# Autodesk Inventor assembly: Ensamble NotAFarmBot2
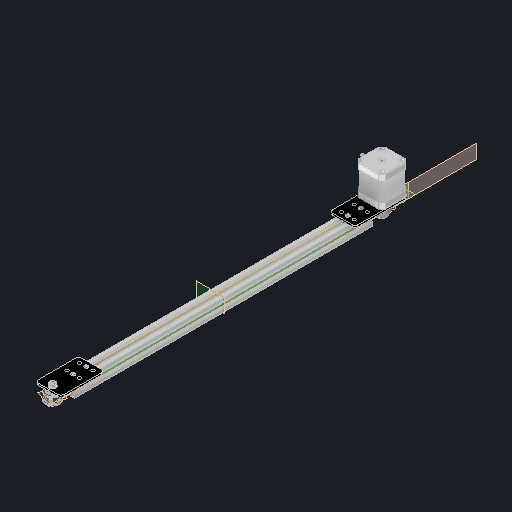
[picture p0: Inventor's stored thumbnail of the model, 512x512]
Saved by Autodesk Inventor 2024 (Build 280153000, 153)
## iProperties
Created: 2020-07-22
Part Number: Ensamble NotAFarmBot2
Document SubType Name: Assembly
Designer: juanp
Mass: 1932.13 g
Surface Area: 7509.2 cm^2
Volume: 1044.57 cm^3
Density: 1.84968 g/cm^3
Author: juanp
## Documents named in this file (17)
- C:\Users\juanp\OneDrive - Universidad de los andes\Uniandes\Robocol\SyE - EVA + RAMSES\EVA\Recursos\Actuador Lineal\Actuador Lineal (sin carro).iam
- C:\Users\juanp\OneDrive - Universidad de los andes\Uniandes\Robocol\SyE - EVA + RAMSES\EVA\Recursos\Actuador Lineal\Partes\VSLOT 2020 Extrusion.ipt
- C:\Users\juanp\OneDrive - Universidad de los andes\Uniandes\Robocol\SyE - EVA + RAMSES\EVA\Recursos\Actuador Lineal\Tornillos-Arandelas-Tuercas-Espaciadores\Double Tee Nut.ipt
- C:\Users\juanp\OneDrive - Universidad de los andes\Uniandes\Robocol\SyE - EVA + RAMSES\EVA\Recursos\Actuador Lineal\Partes\GT2_30T_5_6.ipt
- C:\Users\juanp\OneDrive - Universidad de los andes\Uniandes\Robocol\SyE - EVA + RAMSES\EVA\Recursos\Actuador Lineal\Partes\Idler Pulley Plate.ipt
- C:\Users\juanp\OneDrive - Universidad de los andes\Uniandes\Robocol\SyE - EVA + RAMSES\EVA\Recursos\Actuador Lineal\Partes\Motor Mount Plate Nema 17.ipt
- C:\Users\juanp\OneDrive - Universidad de los andes\Uniandes\Robocol\SyE - EVA + RAMSES\EVA\Recursos\Actuador Lineal\Partes\M1173041- NEMA 17.ipt
- C:\Users\juanp\OneDrive - Universidad de los andes\Uniandes\Robocol\SyE - EVA + RAMSES\EVA\Recursos\Actuador Lineal\Tornillos-Arandelas-Tuercas-Espaciadores\3mm Spacer.ipt
- C:\Users\juanp\OneDrive - Universidad de los andes\Uniandes\Robocol\SyE - EVA + RAMSES\EVA\Recursos\Actuador Lineal\Partes\Ball Bearing 625 2RS 5x16x5.ipt
- C:\Users\juanp\OneDrive - Universidad de los andes\Uniandes\Robocol\SyE - EVA + RAMSES\EVA\Recursos\Actuador Lineal\Tornillos-Arandelas-Tuercas-Espaciadores\1mm 5mm shim.ipt
- C:\Users\juanp\OneDrive - Universidad de los andes\Uniandes\Robocol\SyE - EVA + RAMSES\EVA\Recursos\Actuador Lineal\Tornillos-Arandelas-Tuercas-Espaciadores\Nylon Spacer 1_8th.ipt
- C:\Users\juanp\OneDrive - Universidad de los andes\Uniandes\Robocol\SyE - EVA + RAMSES\EVA\Recursos\Actuador Lineal\Partes\idler pulley.ipt
- C:\Users\juanp\OneDrive - Universidad de los andes\Uniandes\Robocol\SyE - EVA + RAMSES\EVA\Recursos\Actuador Lineal\Tornillos-Arandelas-Tuercas-Espaciadores\M5 Nylock.ipt
- C:\Users\juanp\OneDrive - Universidad de los andes\Uniandes\Robocol\SyE - EVA + RAMSES\EVA\Recursos\Actuador Lineal\Tornillos-Arandelas-Tuercas-Espaciadores\M5x25 low profile screw.ipt
- C:\Users\juanp\Documents\Inventor\Content Center Files\R2020\en-US\ANSI B18.3.1M(1)\ANSI B18.3.1M - M3x0.5 x 8(2).ipt
- C:\Users\juanp\Documents\Inventor\Content Center Files\R2020\en-US\ANSI B18.22 M\ANSI B18.22M - 3 N.ipt
- C:\Users\juanp\Documents\Inventor\Content Center Files\R2020\en-US\ANSI B18.3.4M(2)\ANSI B18.3.4M - M3 x 0.5 x 8(1).ipt
## Components (27 placed, 16 different names)
1. VSLOT 2020 Extrusion:1 — Mate:85, Mate:87, Mate:88, Angle:16, Mate:98, Mate:99, Angle:18, Mate:101, Mate:185, Angle:24, Flush:3, Mate:196, Mate:197, Flush:4, Flush:5
2. Double Tee Nut:1 — Mate:98, Mate:99, Angle:18, Mate:198, Mate:199, Flush:5
3. Double Tee Nut:2 — Mate:85, Mate:87, Angle:16, Mate:200, Mate:201, Flush:4
4. GT2_30T_5_6:2 — Mate:35, Mate:107
5. Idler Pulley Plate:1 — Mate:88, Mate:95, Mate:97, Angle:17, Mate:200, Mate:201, Mate:206, Mate:221, Mate:222
6. Motor Mount Plate Nema 17:1 — Mate:12, Mate:13, Angle:4, Mate:101, Angle:24, Mate:198, Mate:199, Mate:214, Mate:218, Mate:219, Mate:220
7. M1173041- NEMA 17:1 — Mate:12, Mate:13, Angle:4, Mate:107, Mate:213, Mate:215, Mate:216, Mate:217
8. Ball Bearing 625 2RS 5x16x5:1 — Mate:22, Mate:23, Mate:24, Mate:26, Mate:32, Mate:202
9. Ball Bearing 625 2RS 5x16x5:2 — Mate:21, Mate:25, Mate:207
10. 1mm 5mm shim:1 — Mate:47, Mate:97, Mate:205
11. Nylon Spacer 1_8th:1 — Mate:23, Mate:24, Mate:25
12. idler pulley:1 — Mate:21, Mate:22, Mate:26, Mate:35
13. 3mm Spacer:1 — Mate:32, Mate:95, Mate:203
14. M5 Nylock:1 — Mate:47, Angle:17, Mate:204
15. M5x25 low profile screw:1 — Mate:202, Mate:203, Mate:204, Mate:205, Mate:206, Mate:207
16. Broached Socket Head Cap Screw - Metric M3x0.5 x 8:1 — Mate:211, Flush:7, Flush:8, Mate:217
17. Broached Socket Head Cap Screw - Metric M3x0.5 x 8:2 — Mate:210, Flush:8, Mate:212, Mate:216
18. Broached Socket Head Cap Screw - Metric M3x0.5 x 8:3 — Mate:208, Flush:6, Mate:213
19. Broached Socket Head Cap Screw - Metric M3x0.5 x 8:4 — Mate:209, Flush:6, Flush:7, Mate:215
20. Plain Washer (Metric) 3 N:1 — Mate:209, Flush:10, Flush:11, Mate:212, Mate:214
21. Plain Washer (Metric) 3 N:2 — Mate:210, Flush:9
22. Plain Washer (Metric) 3 N:3 — Mate:208, Flush:11
23. Plain Washer (Metric) 3 N:4 — Mate:211, Flush:9, Flush:10
24. Forged Hexagon Socket Button Head Cap Screw - Metric M3 x 0.5 x 8:1 — Flush:12, Mate:222
25. Forged Hexagon Socket Button Head Cap Screw - Metric M3 x 0.5 x 8:2 — Flush:12, Flush:13, Mate:221
26. Forged Hexagon Socket Button Head Cap Screw - Metric M3 x 0.5 x 8:3 — Flush:13, Flush:14, Mate:220
27. Forged Hexagon Socket Button Head Cap Screw - Metric M3 x 0.5 x 8:4 — Flush:14, Mate:218, Mate:219
## Relationships (65: Mate 48, Flush 12, Angle 5)
- Mate:12: Motor Mount Plate Nema 17:1 ↔ M1173041- NEMA 17:1
- Mate:13: Motor Mount Plate Nema 17:1 ↔ M1173041- NEMA 17:1
- Angle:4 (0 deg): Motor Mount Plate Nema 17:1 ↔ M1173041- NEMA 17:1
- Mate:21: Ball Bearing 625 2RS 5x16x5:2 ↔ idler pulley:1
- Mate:22: Ball Bearing 625 2RS 5x16x5:1 ↔ idler pulley:1
- Mate:23: Ball Bearing 625 2RS 5x16x5:1 ↔ Nylon Spacer 1_8th:1
- Mate:24: Ball Bearing 625 2RS 5x16x5:1 ↔ Nylon Spacer 1_8th:1
- Mate:25: Ball Bearing 625 2RS 5x16x5:2 ↔ Nylon Spacer 1_8th:1
- Mate:26: Ball Bearing 625 2RS 5x16x5:1 ↔ idler pulley:1
- Mate:32: Ball Bearing 625 2RS 5x16x5:1 ↔ 3mm Spacer:1
- Mate:35: GT2_30T_5_6:2 ↔ idler pulley:1
- Mate:47: 1mm 5mm shim:1 ↔ M5 Nylock:1
- Mate:85: VSLOT 2020 Extrusion:1 ↔ Double Tee Nut:2
- Mate:87: VSLOT 2020 Extrusion:1 ↔ Double Tee Nut:2
- Mate:88: VSLOT 2020 Extrusion:1 ↔ Idler Pulley Plate:1
- Angle:16 (180 deg): VSLOT 2020 Extrusion:1 ↔ Double Tee Nut:2
- Mate:95: Idler Pulley Plate:1 ↔ 3mm Spacer:1
- Mate:97: Idler Pulley Plate:1 ↔ 1mm 5mm shim:1
- Angle:17 (0 deg): Idler Pulley Plate:1 ↔ M5 Nylock:1
- Mate:98: VSLOT 2020 Extrusion:1 ↔ Double Tee Nut:1
- Mate:99: VSLOT 2020 Extrusion:1 ↔ Double Tee Nut:1
- Angle:18 (0 deg): VSLOT 2020 Extrusion:1 ↔ Double Tee Nut:1
- Mate:101: VSLOT 2020 Extrusion:1 ↔ Motor Mount Plate Nema 17:1
- Mate:107: GT2_30T_5_6:2 ↔ M1173041- NEMA 17:1
- Mate:185: VSLOT 2020 Extrusion:1
- Angle:24 (0 deg): VSLOT 2020 Extrusion:1 ↔ Motor Mount Plate Nema 17:1
- Flush:3: VSLOT 2020 Extrusion:1
- Mate:196: VSLOT 2020 Extrusion:1
- Mate:197: VSLOT 2020 Extrusion:1
- Mate:198: Double Tee Nut:1 ↔ Motor Mount Plate Nema 17:1
- Mate:199: Double Tee Nut:1 ↔ Motor Mount Plate Nema 17:1
- Mate:200: Double Tee Nut:2 ↔ Idler Pulley Plate:1
- Mate:201: Double Tee Nut:2 ↔ Idler Pulley Plate:1
- Mate:202: Ball Bearing 625 2RS 5x16x5:1 ↔ M5x25 low profile screw:1
- Mate:203: 3mm Spacer:1 ↔ M5x25 low profile screw:1
- Mate:204: M5 Nylock:1 ↔ M5x25 low profile screw:1
- Mate:205: 1mm 5mm shim:1 ↔ M5x25 low profile screw:1
- Mate:206: Idler Pulley Plate:1 ↔ M5x25 low profile screw:1
- Flush:4: VSLOT 2020 Extrusion:1 ↔ Double Tee Nut:2
- Flush:5: VSLOT 2020 Extrusion:1 ↔ Double Tee Nut:1
- Mate:207: Ball Bearing 625 2RS 5x16x5:2 ↔ M5x25 low profile screw:1
- Mate:208: Broached Socket Head Cap Screw - Metric M3x0.5 x 8:3 ↔ Plain Washer (Metric) 3 N:3
- Mate:209: Broached Socket Head Cap Screw - Metric M3x0.5 x 8:4 ↔ Plain Washer (Metric) 3 N:1
- Mate:210: Broached Socket Head Cap Screw - Metric M3x0.5 x 8:2 ↔ Plain Washer (Metric) 3 N:2
- Mate:211: Broached Socket Head Cap Screw - Metric M3x0.5 x 8:1 ↔ Plain Washer (Metric) 3 N:4
- Flush:6: Broached Socket Head Cap Screw - Metric M3x0.5 x 8:3 ↔ Broached Socket Head Cap Screw - Metric M3x0.5 x 8:4
- Flush:7: Broached Socket Head Cap Screw - Metric M3x0.5 x 8:1 ↔ Broached Socket Head Cap Screw - Metric M3x0.5 x 8:4
- Flush:8: Broached Socket Head Cap Screw - Metric M3x0.5 x 8:1 ↔ Broached Socket Head Cap Screw - Metric M3x0.5 x 8:2
- Flush:9: Plain Washer (Metric) 3 N:2 ↔ Plain Washer (Metric) 3 N:4
- Flush:10: Plain Washer (Metric) 3 N:1 ↔ Plain Washer (Metric) 3 N:4
- Flush:11: Plain Washer (Metric) 3 N:1 ↔ Plain Washer (Metric) 3 N:3
- Mate:212: Broached Socket Head Cap Screw - Metric M3x0.5 x 8:2 ↔ Plain Washer (Metric) 3 N:1
- Mate:213: M1173041- NEMA 17:1 ↔ Broached Socket Head Cap Screw - Metric M3x0.5 x 8:3
- Mate:214: Motor Mount Plate Nema 17:1 ↔ Plain Washer (Metric) 3 N:1
- Mate:215: M1173041- NEMA 17:1 ↔ Broached Socket Head Cap Screw - Metric M3x0.5 x 8:4
- Mate:216: M1173041- NEMA 17:1 ↔ Broached Socket Head Cap Screw - Metric M3x0.5 x 8:2
- Mate:217: M1173041- NEMA 17:1 ↔ Broached Socket Head Cap Screw - Metric M3x0.5 x 8:1
- Flush:12: Forged Hexagon Socket Button Head Cap Screw - Metric M3 x 0.5 x 8:1 ↔ Forged Hexagon Socket Button Head Cap Screw - Metric M3 x 0.5 x 8:2
- Flush:13: Forged Hexagon Socket Button Head Cap Screw - Metric M3 x 0.5 x 8:2 ↔ Forged Hexagon Socket Button Head Cap Screw - Metric M3 x 0.5 x 8:3
- Flush:14: Forged Hexagon Socket Button Head Cap Screw - Metric M3 x 0.5 x 8:3 ↔ Forged Hexagon Socket Button Head Cap Screw - Metric M3 x 0.5 x 8:4
- Mate:218: Motor Mount Plate Nema 17:1 ↔ Forged Hexagon Socket Button Head Cap Screw - Metric M3 x 0.5 x 8:4
- Mate:219: Motor Mount Plate Nema 17:1 ↔ Forged Hexagon Socket Button Head Cap Screw - Metric M3 x 0.5 x 8:4
- Mate:220: Motor Mount Plate Nema 17:1 ↔ Forged Hexagon Socket Button Head Cap Screw - Metric M3 x 0.5 x 8:3
- Mate:221: Idler Pulley Plate:1 ↔ Forged Hexagon Socket Button Head Cap Screw - Metric M3 x 0.5 x 8:2
- Mate:222: Idler Pulley Plate:1 ↔ Forged Hexagon Socket Button Head Cap Screw - Metric M3 x 0.5 x 8:1
